# Autodesk Inventor assembly: VersaPlanetary_v2_2 Stage_10_1_with_NEO 550_180 deg drive
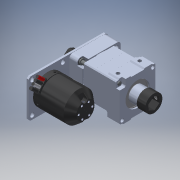
[picture p0: Inventor's stored thumbnail of the model, 180x180]
Saved by Autodesk Inventor 2018.3 (Build 223284000, 284)
## iProperties
Created: 2016-10-31
Part Number: VersaPlanetary_v2_2 Stage_10_1_with_NEO 550_180 deg drive
Description: STEP AP214
Document SubType Name: Assembly
Designer: carls
Sending System: SolidWorks 2016
Preprocessor: SwSTEP 2.0
Title: 217-4973_1stage_550.STEP
Revision Number: ANY
## Documents named in this file (16)
- C:\Users\carls\Documents\GrabCAD\Infinite Recharge 2020\Build season\VersaPlanetary_v2_2 Stage_10_1_with_NEO 550_180 deg drive.iam
- C:\Users\carls\Documents\GrabCAD\Infinite Recharge 2020\Build season\217-2625-026 Rev1.ipt
- C:\Users\carls\Documents\GrabCAD\Infinite Recharge 2020\Build season\217-2742-001 Rev4.ipt
- C:\Users\carls\Documents\GrabCAD\Infinite Recharge 2020\Build season\217-2625-017 Rev1_9714K61.ipt
- C:\Users\carls\Documents\GrabCAD\Infinite Recharge 2020\Build season\217-2625-018 Rev1_98541A410.ipt
- C:\Users\carls\Documents\GrabCAD\Infinite Recharge 2020\Build season\832-1750-Ring-Gear-Screw_SSA0832-0500ZC.ipt
- C:\Users\carls\Documents\GrabCAD\Infinite Recharge 2020\Build season\217-4649-005 Rev1_SSA0003-008BA.ipt
- C:\Users\carls\Documents\GrabCAD\Infinite Recharge 2020\Build season\217-2820 Rev1_Public.iam
- C:\Users\carls\Documents\GrabCAD\Infinite Recharge 2020\Build season\217-2816-001 Rev1.ipt
- C:\Users\carls\Documents\GrabCAD\Infinite Recharge 2020\Build season\217-4649-001 Rev1.ipt
- C:\Users\carls\Documents\GrabCAD\Infinite Recharge 2020\Build season\217-4649-007 Rev1_94105A824.ipt
- C:\Users\carls\Documents\GrabCAD\Infinite Recharge 2020\Build season\217-2625-012 Rev1.ipt
- C:\Users\carls\Documents\GrabCAD\Infinite Recharge 2020\Build season\Universal_Female_Output_Shaft_1_2_Hex_.iam
- C:\Users\carls\Documents\GrabCAD\Infinite Recharge 2020\Build season\REV Neo 550.ipt
- C:\Users\carls\Documents\GrabCAD\Infinite Recharge 2020\Build season\VersaPlanetary_180_Drive_Gusset_Kit (1).ipt
- C:\Users\carls\Documents\GrabCAD\Infinite Recharge 2020\Build season\VersaPlanetary_180_Drive_-_Speed_Reducer (1).iam
## Components (18 placed, 18 different names)
1. 217-2625-026 Rev1_1 — Insert:1, Flush:1
2. 217-2742-001 Rev4_2
3. 217-2742-001 Rev4_3 — Insert:5
4. 217-2625-017 Rev1_9714K61_4
5. 217-2625-018 Rev1_98541A410_6
6. 832-1750-Ring-Gear-Screw_SSA0832-0500ZC_7
7. 832-1750-Ring-Gear-Screw_SSA0832-0500ZC_8
8. 217-4649-005 Rev1_SSA0003-008BA_12
9. 217-2820 Rev1_Public_16 [sub-assembly]
10. 217-2816-001 Rev1_17 — Insert:1, Flush:1, Insert:2, Flush:2
11. 217-4649-001 Rev1_18
12. 217-4649-007 Rev1_94105A824_19
13. 217-2625-012 Rev1_20
14. 217-2816-001 Rev1:2 — Insert:2, Flush:2, Insert:9
15. Universal_Female_Output_Shaft_1_2_Hex_:1 [sub-assembly] — Insert:5
16. REV Neo 550:1 — Insert:11
17. VersaPlanetary_180_Drive_Gusset_Kit (1):1 — Insert:10, Insert:11
18. VersaPlanetary_180_Drive_-_Speed_Reducer (1):1 [sub-assembly] — Insert:9, Insert:10
## Relationships (8: Insert 6, Flush 2)
- Insert:1: 217-2625-026 Rev1_1 ↔ 217-2816-001 Rev1_17
- Flush:1: 217-2625-026 Rev1_1 ↔ 217-2816-001 Rev1_17
- Insert:2: 217-2816-001 Rev1_17 ↔ 217-2816-001 Rev1:2
- Flush:2: 217-2816-001 Rev1_17 ↔ 217-2816-001 Rev1:2
- Insert:5: 217-2742-001 Rev4_3 ↔ Universal_Female_Output_Shaft_1_2_Hex_:1
- Insert:9: 217-2816-001 Rev1:2 ↔ VersaPlanetary_180_Drive_-_Speed_Reducer (1):1
- Insert:10: VersaPlanetary_180_Drive_Gusset_Kit (1):1 ↔ VersaPlanetary_180_Drive_-_Speed_Reducer (1):1
- Insert:11: REV Neo 550:1 ↔ VersaPlanetary_180_Drive_Gusset_Kit (1):1
